# Autodesk Inventor assembly: LEG_MIR_MIR1_MIR
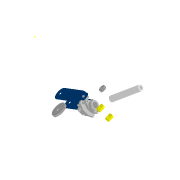
[picture p0: Inventor's stored thumbnail of the model, 180x180]
Saved by Autodesk Inventor 2020.5 (Build 245400000, 400)
## iProperties
Created: 2022-10-31
Part Number: LEG_MIR_MIR1_MIR
Document SubType Name: Assembly
Designer: Administrator
Author: Administrator
## Documents named in this file (12)
- C:\Users\Administrator\Documents\kamuy2\kamuy2\LEG_MIR_MIR1_MIR.iam
- C:\Users\Administrator\Documents\kamuy2\kamuy2\Parts\Part2_MIR_MIR_MIR1_MIR.ipt
- C:\Users\Administrator\Documents\kamuy2\kamuy2\Parts\GEABP1.0-70-10-A-19-KFC30-K3_Autodesk_Inventor_2020_20221114\AIS2020\GEABP1_0-70-10-A-19-KFC30-K3_MIR_MIR_MIR1_MIR.iam
- C:\Users\Administrator\Documents\kamuy2\kamuy2\Parts\PIJX30-20-150_Autodesk_Inventor_2020_20221115\PIJX30-20-150_MIR_MIR_MIR1_MIR.ipt
- C:\Users\Administrator\Documents\kamuy2\kamuy2\Parts\C-SHA10_Autodesk_Inventor_2020_20221104\AIS2020\C-SHA10_MIR_MIR_MIR1_MIR.iam
- C:\Users\Administrator\Documents\kamuy2\kamuy2\Part16_MIR_MIR_MIR1_MIR.ipt
- C:\Users\Administrator\Documents\kamuy2\kamuy2\Parts\HTPA30S3M060-A-N10_Autodesk_Inventor_2020_20221115\AIS2020\HTPA30S3M060-A-N10_MIR_MIR_MIR1_MIR.iam
- C:\Users\Administrator\Documents\kamuy2\kamuy2\Part20_MIR_MIR_MIR1_MIR.ipt
- C:\Users\Administrator\Documents\kamuy2\kamuy2\Parts\SMYHF30_STEP_AP203AP214\SMYHF30_203_MIR_MIR_MIR1_MIR.ipt
- C:\Users\Administrator\Documents\kamuy2\kamuy2\Parts\RORPOS20-L30_Autodesk_Inventor_2020_20221117\AIS2020\RORPOS20-L30_MIR_MIR_MIR1_MIR.iam
- C:\Users\Administrator\Documents\kamuy2\kamuy2\Parts\NSFMRRA10-74-B3-S3-KC31.5-A11_Autodesk_Inventor_2020_20221116\AIS2020\NSFMRRA10-74-B3-S3-KC31_5-A11(000_000)_MIR_MIR_MIR1_MIR.iam
- C:\Users\Administrator\Documents\kamuy2\kamuy2\3dprinter\Part77.ipt
## Components (16 placed, 11 different names)
1. Part2_MIR_MIR_MIR1_MIR:1
2. GEABP1_0-70-10-A-19-KFC30-K3_MIR_MIR_MIR1_MIR:1 [sub-assembly] — フラッシュ:123
3. PIJX30-20-150_MIR_MIR_MIR1_MIR:1 — メイト:244, メイト:24
4. C-SHA10_MIR_MIR_MIR1_MIR:1 [sub-assembly] — フラッシュ:89, フラッシュ:131, メイト:235, メイト:264
5. C-SHA10_MIR_MIR_MIR1_MIR:2 [sub-assembly] — フラッシュ:89, フラッシュ:131, メイト:237, フラッシュ:10, メイト:23, フラッシュ:11
6. Part16_MIR_MIR_MIR1_MIR:1 — フラッシュ:96, フラッシュ:122, メイト:236
7. Part16_MIR_MIR_MIR1_MIR:2 — フラッシュ:96, メイト:219, メイト:164, メイト:230, メイト:25
8. Part16_MIR_MIR_MIR1_MIR:3 — メイト:219, フラッシュ:122, メイト:234, フラッシュ:139, メイト:26
9. HTPA30S3M060-A-N10_MIR_MIR_MIR1_MIR:1 [sub-assembly] — フラッシュ:138, メイト:263
10. HTPA30S3M060-A-N10_MIR_MIR_MIR1_MIR:2 [sub-assembly] — メイト:164, フラッシュ:138
11. Part20_MIR_MIR_MIR1_MIR:1 — フラッシュ:123, メイト:236, メイト:237, メイト:265, メイト:68, メイト:66
12. Part20_MIR_MIR_MIR1_MIR:2 — メイト:230, メイト:234, メイト:235, メイト:265, メイト:247, メイト:251, メイト:69, メイト:253
13. SMYHF30_203_MIR_MIR_MIR1_MIR:1 — メイト:244, メイト:23, フラッシュ:11
14. RORPOS20-L30_MIR_MIR_MIR1_MIR:1 [sub-assembly] — メイト:247, メイト:251
15. NSFMRRA10-74-B3-S3-KC31_5-A11(000_000)_MIR_MIR_MIR1_MIR:1 [sub-assembly] — メイト:69, メイト:68, メイト:66, フラッシュ:139, メイト:253, メイト:263, メイト:264, メイト:25, メイト:26
16. Part77:1 — フラッシュ:10, メイト:24
## Relationships (30: Mate 21, Flush 9)
- フラッシュ:89 [Flush]: C-SHA10_MIR_MIR_MIR1_MIR:1 ↔ C-SHA10_MIR_MIR_MIR1_MIR:2
- フラッシュ:131 [Flush]: C-SHA10_MIR_MIR_MIR1_MIR:1 ↔ C-SHA10_MIR_MIR_MIR1_MIR:2
- フラッシュ:96 [Flush]: Part16_MIR_MIR_MIR1_MIR:1 ↔ Part16_MIR_MIR_MIR1_MIR:2
- メイト:219 [Mate] (168 mm): Part16_MIR_MIR_MIR1_MIR:2 ↔ Part16_MIR_MIR_MIR1_MIR:3
- フラッシュ:122 [Flush]: Part16_MIR_MIR_MIR1_MIR:1 ↔ Part16_MIR_MIR_MIR1_MIR:3
- メイト:164 [Mate] (7 mm): Part16_MIR_MIR_MIR1_MIR:2 ↔ HTPA30S3M060-A-N10_MIR_MIR_MIR1_MIR:2
- フラッシュ:138 [Flush]: HTPA30S3M060-A-N10_MIR_MIR_MIR1_MIR:1 ↔ HTPA30S3M060-A-N10_MIR_MIR_MIR1_MIR:2
- フラッシュ:123 [Flush]: GEABP1_0-70-10-A-19-KFC30-K3_MIR_MIR_MIR1_MIR:1 ↔ Part20_MIR_MIR_MIR1_MIR:1
- メイト:236 [Mate]: Part16_MIR_MIR_MIR1_MIR:1 ↔ Part20_MIR_MIR_MIR1_MIR:1
- メイト:237 [Mate] (6 mm): C-SHA10_MIR_MIR_MIR1_MIR:2 ↔ Part20_MIR_MIR_MIR1_MIR:1
- メイト:230 [Mate]: Part16_MIR_MIR_MIR1_MIR:2 ↔ Part20_MIR_MIR_MIR1_MIR:2
- メイト:234 [Mate]: Part16_MIR_MIR_MIR1_MIR:3 ↔ Part20_MIR_MIR_MIR1_MIR:2
- メイト:235 [Mate] (6 mm): C-SHA10_MIR_MIR_MIR1_MIR:1 ↔ Part20_MIR_MIR_MIR1_MIR:2
- メイト:265 [Mate]: Part20_MIR_MIR_MIR1_MIR:1 ↔ Part20_MIR_MIR_MIR1_MIR:2
- メイト:244 [Mate]: PIJX30-20-150_MIR_MIR_MIR1_MIR:1 ↔ SMYHF30_203_MIR_MIR_MIR1_MIR:1
- メイト:247 [Mate] (2.5 mm): Part20_MIR_MIR_MIR1_MIR:2 ↔ RORPOS20-L30_MIR_MIR_MIR1_MIR:1
- メイト:251 [Mate]: Part20_MIR_MIR_MIR1_MIR:2 ↔ RORPOS20-L30_MIR_MIR_MIR1_MIR:1
- メイト:69 [Mate]: Part20_MIR_MIR_MIR1_MIR:2 ↔ NSFMRRA10-74-B3-S3-KC31_5-A11(000_000)_MIR_MIR_MIR1_MIR:1
- メイト:68 [Mate]: Part20_MIR_MIR_MIR1_MIR:1 ↔ NSFMRRA10-74-B3-S3-KC31_5-A11(000_000)_MIR_MIR_MIR1_MIR:1
- メイト:66 [Mate]: Part20_MIR_MIR_MIR1_MIR:1 ↔ NSFMRRA10-74-B3-S3-KC31_5-A11(000_000)_MIR_MIR_MIR1_MIR:1
- フラッシュ:139 [Flush] (-3 mm): Part16_MIR_MIR_MIR1_MIR:3 ↔ NSFMRRA10-74-B3-S3-KC31_5-A11(000_000)_MIR_MIR_MIR1_MIR:1
- メイト:253 [Mate]: Part20_MIR_MIR_MIR1_MIR:2 ↔ NSFMRRA10-74-B3-S3-KC31_5-A11(000_000)_MIR_MIR_MIR1_MIR:1
- メイト:263 [Mate]: HTPA30S3M060-A-N10_MIR_MIR_MIR1_MIR:1 ↔ NSFMRRA10-74-B3-S3-KC31_5-A11(000_000)_MIR_MIR_MIR1_MIR:1
- メイト:264 [Mate]: C-SHA10_MIR_MIR_MIR1_MIR:1 ↔ NSFMRRA10-74-B3-S3-KC31_5-A11(000_000)_MIR_MIR_MIR1_MIR:1
- フラッシュ:10 [Flush]: C-SHA10_MIR_MIR_MIR1_MIR:2 ↔ Part77:1
- メイト:23 [Mate] (15 mm): C-SHA10_MIR_MIR_MIR1_MIR:2 ↔ SMYHF30_203_MIR_MIR_MIR1_MIR:1
- フラッシュ:11 [Flush] (-20 mm): C-SHA10_MIR_MIR_MIR1_MIR:2 ↔ SMYHF30_203_MIR_MIR_MIR1_MIR:1
- メイト:24 [Mate]: PIJX30-20-150_MIR_MIR_MIR1_MIR:1 ↔ Part77:1
- メイト:25 [Mate]: Part16_MIR_MIR_MIR1_MIR:2 ↔ NSFMRRA10-74-B3-S3-KC31_5-A11(000_000)_MIR_MIR_MIR1_MIR:1
- メイト:26 [Mate]: Part16_MIR_MIR_MIR1_MIR:3 ↔ NSFMRRA10-74-B3-S3-KC31_5-A11(000_000)_MIR_MIR_MIR1_MIR:1
